# Autodesk Inventor assembly: Shock Body
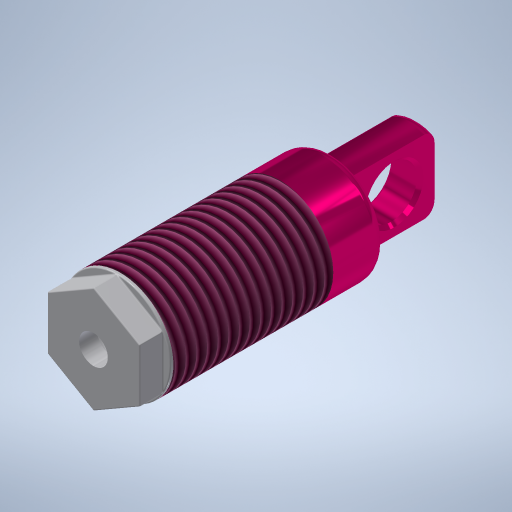
[picture p0: Inventor's stored thumbnail of the model, 512x512]
Saved by Autodesk Inventor 2023.1 (Build 271208000, 208)
## iProperties
Created: 2019-12-02
Part Number: Shock Body
Document SubType Name: Assembly
Designer: Jopa
Author: Jopa
## Documents named in this file (3)
- C:\Users\Arzum Naz Doğaner\OneDrive\Masaüstü\HUDSON süspansiyon\Shock Body.iam
- C:\Users\Arzum Naz Doğaner\OneDrive\Masaüstü\HUDSON süspansiyon\Shock Body 1.3 Length.ipt
- C:\Users\Arzum Naz Doğaner\OneDrive\Masaüstü\HUDSON süspansiyon\Shock Cartridge.iam
## Components (2 placed, 2 different names)
1. Shock Body 1.3 Length:1 — Mate:1, Mate:2, Angle:1
2. Shock Cartridge:1 [sub-assembly] — Mate:1, Mate:2, Angle:1
## Relationships (3: Mate 2, Angle 1)
- Mate:1: Shock Body 1.3 Length:1 ↔ Shock Cartridge:1
- Mate:2: Shock Body 1.3 Length:1 ↔ Shock Cartridge:1
- Angle:1 (0 deg): Shock Body 1.3 Length:1 ↔ Shock Cartridge:1
